# Autodesk Inventor assembly: UBG-Dribblerhalter v2
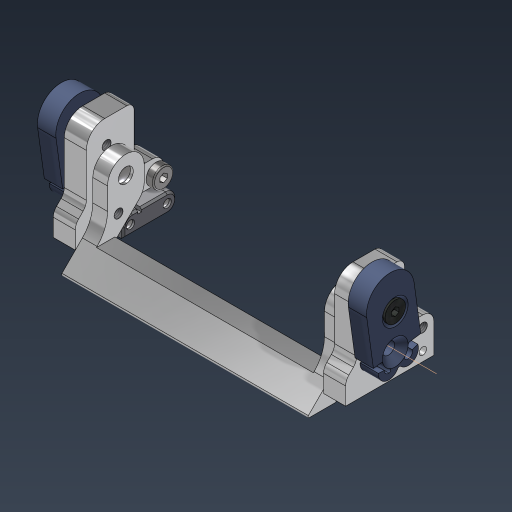
[picture p0: Inventor's stored thumbnail of the model, 512x512]
Saved by Autodesk Inventor 2023.1 (Build 271208000, 208)
## iProperties
Part Number: UBG-Dribblerhalter v2
Material: Generisch
Document SubType Name: Assembly
Designer: rYan
Mass: 57.0312 g
Surface Area: 178.036 cm^2
Volume: 20.8384 cm^3
Density: 2.73684 g/cm^3
Author: rYan
## Documents named in this file (13)
- D:\TIGERsGIT\Hardware\mechanik\2024\Inventor\Robot\Dribbler\UBG-Dribblerhalter v2.iam
- D:\TIGERsGIT\Hardware\mechanik\2024\Inventor\Inhaltscenter\de-DE\ISO 8745(2)\ISO 8745 - 4 x 10(6).ipt
- D:\TIGERsGIT\Hardware\mechanik\2024\Inventor\Purchased Parts\Zugfeder RZ-006DI.ipt
- D:\TIGERsGIT\Hardware\mechanik\2024\Inventor\Inhaltscenter\de-DE\DIN 7984\DIN 7984 - M3 x 5.ipt
- D:\TIGERsGIT\Hardware\mechanik\2024\Inventor\Purchased Parts\ISO 10642 - M3 x  6.ipt
- D:\TIGERsGIT\Hardware\mechanik\2024\Inventor\Robot\Dribbler\Dribbler Lagerbock v2.ipt
- D:\TIGERsGIT\Hardware\mechanik\2024\Inventor\Inhaltscenter\de-DE\ISO 8745(2)\ISO 8745 - 2 x 10(6).ipt
- D:\TIGERsGIT\Hardware\mechanik\2024\Inventor\Robot\Kicker\MG-Chip Schaufel.iam
- D:\TIGERsGIT\Hardware\mechanik\2024\Inventor\Inhaltscenter\de-DE\ISO 10642(1)\ISO 10642 - M3 x  8.ipt
- D:\TIGERsGIT\Hardware\mechanik\2024\Inventor\Robot\Dribbler\Dribbler Slider.ipt
- D:\TIGERsGIT\Hardware\mechanik\2024\Inventor\Robot\Kicker\Chip Schaufel v2.ipt
- D:\TIGERsGIT\Hardware\mechanik\2024\Inventor\Robot\Dribbler\Chipanschlag L2.0.ipt
- D:\TIGERsGIT\Hardware\mechanik\2024\Inventor\Robot\Dribbler\Dribbler Slider gespiegelt.ipt
## Components (19 placed, 12 different names)
1. Dribbler Lagerbock v2:3 — Passend:2, Passend:4, Symmetrie:1, Passend:5, Einfügen:4, Passend:6, Winkel:1, Einfügen:5, Einfügen:19, Einfügen:20, Winkel:2, Einfügen:32, Einfügen:34, Passend:23
2. Dribbler Lagerbock v2:4 — Passend:1, Passend:3, Symmetrie:1, Passend:5, Einfügen:3, Einfügen:6, Passend:12, Passend:17, Passend:18, Einfügen:33, Passend:22
3. DIN EN ISO 8745 4 x 10:3 — Einfügen:4
4. DIN EN ISO 8745 4 x 10:4 — Einfügen:3
5. Chip Schaufel v2:1 — Passend:6, Fluchtend:1, Winkel:1, Einfügen:9, Einfügen:10
6. Zugfeder RZ-006DI:1
7. DIN 7984 M3 x 5:1 — Einfügen:5
8. DIN 7984 M3 x 5:2 — Einfügen:6
9. ISO 10642 M3 x  6:1 — Einfügen:10
10. ISO 10642 M3 x  6:2 — Einfügen:9
11. DIN EN ISO 8745 2 x 10:1 — Einfügen:19
12. DIN EN ISO 8745 2 x 10:2 — Einfügen:20, Passend:21
13. MG-Chip Schaufel:1 [sub-assembly] — Fluchtend:2, Passend:12, Winkel:2
14. ISO 10642 M3 x  8:1
15. ISO 10642 M3 x  8:2
16. Dribbler Slider:2 — Einfügen:33, Passend:22
17. ISO 10642 M3 x  8:3
18. Chipanschlag L2.0:1 — Einfügen:32, Passend:21
19. Dribbler Slider gespiegelt:1 — Einfügen:34, Passend:23
## Relationships (30: Mate 14, Insert 11, Flush 2, Angle 2, Symmetry 1)
- Passend:1 [Mate]: Dribbler Lagerbock v2:4
- Passend:2 [Mate]: Dribbler Lagerbock v2:3
- Passend:3 [Mate]: Dribbler Lagerbock v2:4
- Passend:4 [Mate]: Dribbler Lagerbock v2:3
- Symmetrie:1: Dribbler Lagerbock v2:3 ↔ Dribbler Lagerbock v2:4
- Passend:5 [Mate] (67.5 mm): Dribbler Lagerbock v2:3 ↔ Dribbler Lagerbock v2:4
- Einfügen:3 [Insert] (0.5 mm): Dribbler Lagerbock v2:4 ↔ DIN EN ISO 8745 4 x 10:4
- Einfügen:4 [Insert] (0.5 mm): Dribbler Lagerbock v2:3 ↔ DIN EN ISO 8745 4 x 10:3
- Passend:6 [Mate]: Dribbler Lagerbock v2:3 ↔ Chip Schaufel v2:1
- Fluchtend:1 [Flush]: Chip Schaufel v2:1
- Winkel:1 [Angle] (0 deg): Dribbler Lagerbock v2:3 ↔ Chip Schaufel v2:1
- Einfügen:5 [Insert] (1 mm): Dribbler Lagerbock v2:3 ↔ DIN 7984 M3 x 5:1
- Einfügen:6 [Insert] (1 mm): Dribbler Lagerbock v2:4 ↔ DIN 7984 M3 x 5:2
- Einfügen:9 [Insert]: Chip Schaufel v2:1 ↔ ISO 10642 M3 x  6:2
- Einfügen:10 [Insert]: Chip Schaufel v2:1 ↔ ISO 10642 M3 x  6:1
- Einfügen:19 [Insert]: Dribbler Lagerbock v2:3 ↔ DIN EN ISO 8745 2 x 10:1
- Einfügen:20 [Insert]: Dribbler Lagerbock v2:3 ↔ DIN EN ISO 8745 2 x 10:2
- Fluchtend:2 [Flush]: MG-Chip Schaufel:1
- Passend:12 [Mate]: Dribbler Lagerbock v2:4 ↔ MG-Chip Schaufel:1
- Passend:17 [Mate]: Dribbler Lagerbock v2:4
- Passend:18 [Mate]: Dribbler Lagerbock v2:4
- Passend:19 [Mate]
- Passend:20 [Mate]
- Winkel:2 [Angle] (-3.5 deg): Dribbler Lagerbock v2:3 ↔ MG-Chip Schaufel:1
- Einfügen:32 [Insert]: Dribbler Lagerbock v2:3 ↔ Chipanschlag L2.0:1
- Passend:21 [Mate]: DIN EN ISO 8745 2 x 10:2 ↔ Chipanschlag L2.0:1
- Einfügen:33 [Insert]: Dribbler Lagerbock v2:4 ↔ Dribbler Slider:2
- Passend:22 [Mate]: Dribbler Lagerbock v2:4 ↔ Dribbler Slider:2
- Einfügen:34 [Insert]: Dribbler Lagerbock v2:3 ↔ Dribbler Slider gespiegelt:1
- Passend:23 [Mate]: Dribbler Lagerbock v2:3 ↔ Dribbler Slider gespiegelt:1
